# Autodesk Inventor assembly: WheelMotorAsem
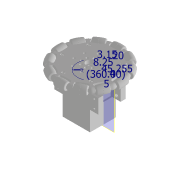
[picture p0: Inventor's stored thumbnail of the model, 180x180]
Saved by Autodesk Inventor 2022 (Build 260153000, 153)
## iProperties
Created: 2022-10-20
Part Number: WheelMotorAsem
Document SubType Name: Assembly
Designer: MVeszpremi
Author: MVeszpremi
## Documents named in this file (4)
- C:\Users\veszp\Dropbox\180DAB CAD\WheelMotorAsem.iam
- C:\Users\veszp\Dropbox\180DAB CAD\StepperWheelConnector.ipt
- C:\Users\veszp\Dropbox\180DAB CAD\StepperMotorHolder.ipt
- C:\Users\veszp\Dropbox\180DAB CAD\Wheel.ipt
## Components (3 placed, 3 different names)
1. StepperWheelConnector:1 — Mate:1, Mate:2
2. StepperMotorHolder:1 — Mate:1, Mate:2
3. Wheel:1
## Relationships (2: Mate 2)
- Mate:1: StepperWheelConnector:1 ↔ StepperMotorHolder:1
- Mate:2 (-3 mm): StepperWheelConnector:1 ↔ StepperMotorHolder:1
